# Autodesk Inventor assembly: full_dog
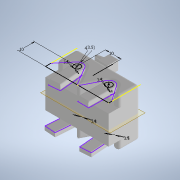
[picture p0: Inventor's stored thumbnail of the model, 180x180]
Saved by Autodesk Inventor 2020 (Build 240168000, 168)
## iProperties
Created: 2020-12-19
Part Number: full_dog
Document SubType Name: Assembly
Designer: frost
Author: frost
## Documents named in this file (4)
- C:\Users\frost\OneDrive\Desktop\Doggy\full_dog.iam
- C:\Users\frost\OneDrive\Desktop\Doggy\dog_body.ipt
- C:\Users\frost\OneDrive\Desktop\Doggy\bog-leg.ipt
- C:\Users\frost\OneDrive\Desktop\Doggy\dog_head.ipt
## Components (6 placed, 3 different names)
1. dog_body:1 — Insert:1, Insert:2, Insert:3, Insert:4, Insert:5
2. bog-leg:2 — Insert:1
3. bog-leg:3 — Insert:2
4. bog-leg:4 — Insert:4
5. bog-leg:5 — Insert:3
6. dog_head:1 — Insert:5
## Relationships (5: Insert 5)
- Insert:1: dog_body:1 ↔ bog-leg:2
- Insert:2: dog_body:1 ↔ bog-leg:3
- Insert:3: dog_body:1 ↔ bog-leg:5
- Insert:4: dog_body:1 ↔ bog-leg:4
- Insert:5: dog_body:1 ↔ dog_head:1
